# Autodesk Inventor assembly: pin1x1
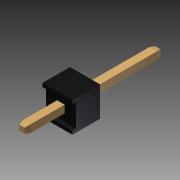
[picture p0: Inventor's stored thumbnail of the model, 180x180]
Saved by Autodesk Inventor 2013 (Build 170138000, 138)
## iProperties
Created: 2016-10-06
Part Number: pin1x1
Document SubType Name: Assembly
Designer: Fede
Author: Fede
## Documents named in this file (3)
- C:\0000 FEDE\16GB\0000 INTERIOR\DE_TMP_BAS\BAS_DTON - demora conexion al energizar\DTON_MANUAL\img\INVENTOR\BAS_DTON_PIN - SIN R\pin1x1.iam
- C:\0000 FEDE\16GB\0000 INTERIOR\DE_TMP_BAS\BAS_DTON - demora conexion al energizar\DTON_MANUAL\img\INVENTOR\BAS_DTON_PIN - SIN R\cgrid 1x1 parte2.ipt
- C:\0000 FEDE\16GB\0000 INTERIOR\DE_TMP_BAS\BAS_DTON - demora conexion al energizar\DTON_MANUAL\img\INVENTOR\BAS_DTON_PIN - SIN R\pin.ipt
## Components (2 placed, 2 different names)
1. cgrid 1x1 parte2:1 — Mate:1, Flush:1, Flush:2, Flush:3
2. pin:1 — Flush:1, Flush:2, Flush:3
## Relationships (4: Flush 3, Mate 1)
- Mate:1: cgrid 1x1 parte2:1
- Flush:1 (-3 mm): cgrid 1x1 parte2:1 ↔ pin:1
- Flush:2: cgrid 1x1 parte2:1 ↔ pin:1
- Flush:3: cgrid 1x1 parte2:1 ↔ pin:1
